# Autodesk Inventor assembly: gusset
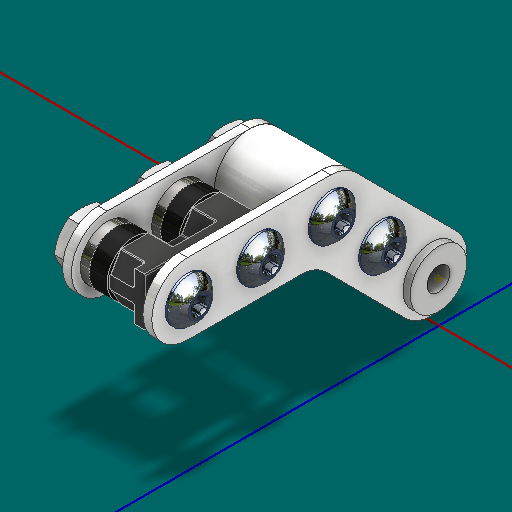
[picture p0: Inventor's stored thumbnail of the model, 512x512]
Saved by Autodesk Inventor 2025 (Build 290162000, 162)
## iProperties
Created: 2024-08-18
Part Number: gusset
Document SubType Name: Assembly
Designer: averey
Author: averey
## Documents named in this file (17)
- C:\Users\avere\vex_robotics_high_stakes\hardware\cad\ATLAS\intake\first_stage\arm\gusset.iam
- C:\Users\avere\vex_robotics_high_stakes\hardware\cad\ATLAS\intake\first_stage\arm\custom_parts\gusset.ipt
- C:\Users\avere\vex_robotics_high_stakes\hardware\cad\VEX-CAD-Inventor\Motion\Spacers\Spacer Nylon .500 OD\NSpacer White .500 OD x .500.ipt
- C:\Users\avere\vex_robotics_high_stakes\hardware\cad\VEX-CAD-Inventor\Motion\Spacers\Spacer Nylon .500 OD.ipt
- C:\Users\avere\vex_robotics_high_stakes\hardware\cad\VEX-CAD-Inventor\Motion\Insert Circle.ipt
- C:\Users\avere\vex_robotics_high_stakes\hardware\cad\VEX-CAD-Inventor\Motion\Spacers\Washer Steel\SWasher .375 OD x .062500.ipt
- C:\Users\avere\vex_robotics_high_stakes\hardware\cad\VEX-CAD-Inventor\Motion\Spacers\Washer Steel.ipt
- C:\Users\avere\vex_robotics_high_stakes\hardware\cad\VEX-CAD-Inventor\Motion\Spacers\Spacer Nylon .375 OD\NSpacer .375 OD x .250.ipt
- C:\Users\avere\vex_robotics_high_stakes\hardware\cad\VEX-CAD-Inventor\Motion\Spacers\Spacer Nylon .375 OD.ipt
- C:\Users\avere\vex_robotics_high_stakes\hardware\cad\VEX-CAD-Inventor\Motion\Spacers\Washer Steel\SWasher .375 OD x .015625.ipt
- C:\Users\avere\vex_robotics_high_stakes\hardware\cad\VEX-CAD-Inventor\Structure\Hardware\Screw Steel - Star\SScrew Star Smooth .750.ipt
- C:\Users\avere\vex_robotics_high_stakes\hardware\cad\VEX-CAD-Inventor\Structure\Hardware\Screw Steel - Star.ipt
- C:\Users\avere\vex_robotics_high_stakes\hardware\cad\custom_parts\modified_parts\Bearing Flat Low Profile 2-Hole.ipt
- C:\Users\avere\vex_robotics_high_stakes\hardware\cad\VEX-CAD-Inventor\Motion\Spacers\Spacer Nylon .375 OD\NSpacer .375 OD x .125.ipt
- C:\Users\avere\vex_robotics_high_stakes\hardware\cad\VEX-CAD-Inventor\Structure\Hardware\Nut Nylon\Nut Nylon - White.ipt
- C:\Users\avere\vex_robotics_high_stakes\hardware\cad\VEX-CAD-Inventor\Structure\Hardware\Nut Nylon.ipt
- C:\Users\avere\vex_robotics_high_stakes\hardware\cad\VEX-CAD-Inventor\Structure\Hardware\Nut Thin Nylock.ipt
## Components (23 placed, 11 different names)
1. gusset:1
2. gusset:2
3. NSpacer White .500 OD x .500:1
4. NSpacer White .500 OD x .500:2
5. Insert Circle:1 — Mate:5
6. Insert Circle:2 — Insert:22
7. SWasher .375 OD x .062500:1
8. SWasher .375 OD x .062500:2
9. NSpacer .375 OD x .250:1
10. SWasher .375 OD x .015625:3
11. SWasher .375 OD x .062500:4
12. SScrew Star Smooth .750:1
13. SScrew Star Smooth .750:2
14. Bearing Flat Low Profile 2-Hole:1
15. NSpacer .375 OD x .125:2
16. NSpacer .375 OD x .125:3
17. Nut Nylon - White:1
18. Nut Nylon - White:2
19. SScrew Star Smooth .750:3
20. Nut Nylon - White:3
21. SScrew Star Smooth .750:4
22. Nut Nylon - White:4
23. Nut Thin Nylock:1 — Insert:22
## Relationships (27: Insert 22, Mate 5)
- [Insert] (12.7 mm): gusset:1 ↔ gusset:2
- [Mate]: gusset:1 ↔ gusset:2
- [Insert]: gusset:1 ↔ NSpacer White .500 OD x .500:1
- [Insert]: gusset:1 ↔ NSpacer White .500 OD x .500:2
- [Insert]: gusset:1 ↔ Insert Circle:1
- [Insert]: gusset:2 ↔ Insert Circle:2
- [Mate]: gusset:2 ↔ Insert Circle:2
- [Mate]: gusset:1 ↔ Insert Circle:1
- [Insert]: gusset:2 ↔ SWasher .375 OD x .062500:1
- [Insert]: gusset:2 ↔ SWasher .375 OD x .062500:2
- [Insert]: SWasher .375 OD x .015625:3 ↔ SWasher .375 OD x .062500:4
- [Insert]: NSpacer .375 OD x .250:1 ↔ SWasher .375 OD x .062500:4
- [Insert]: Insert Circle:2 ↔ NSpacer .375 OD x .250:1
- [Insert]: gusset:1 ↔ SScrew Star Smooth .750:1
- [Insert]: gusset:1 ↔ SScrew Star Smooth .750:2
- [Insert]: SWasher .375 OD x .062500:2 ↔ NSpacer .375 OD x .125:3
- [Insert]: SWasher .375 OD x .062500:1 ↔ NSpacer .375 OD x .125:2
- [Insert]: gusset:2 ↔ Nut Nylon - White:2
- [Insert]: gusset:2 ↔ Nut Nylon - White:1
- [Insert] (15.875 mm): SScrew Star Smooth .750:3 ↔ Nut Nylon - White:3
- [Insert]: gusset:1 ↔ SScrew Star Smooth .750:3
- [Insert] (15.875 mm): SScrew Star Smooth .750:4 ↔ Nut Nylon - White:4
- [Insert]: gusset:1 ↔ SScrew Star Smooth .750:4
- [Insert] (1.27 mm): Bearing Flat Low Profile 2-Hole:1 ↔ NSpacer .375 OD x .125:3
- [Mate]: Bearing Flat Low Profile 2-Hole:1 ↔ NSpacer .375 OD x .125:2
- Mate:5: Insert Circle:1
- Insert:22: Insert Circle:2 ↔ Nut Thin Nylock:1
## Named parameters: d0_d21 = 12.7 mm, d1_d22 = 0 mm, d2_d23 = 0 mm, d3_d24 = 0 mm, d61_d59 = 15.875 mm
